# Autodesk Inventor assembly: Assembly2
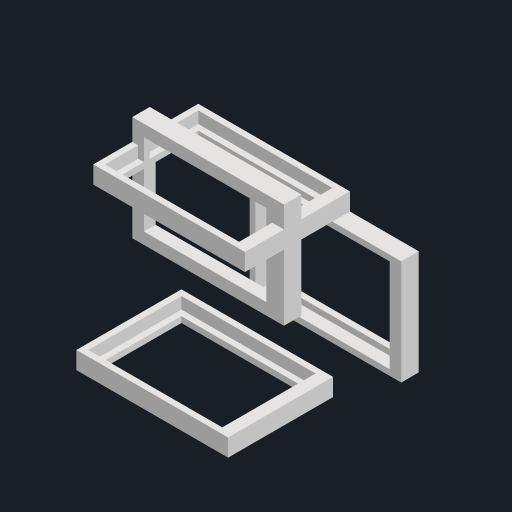
[picture p0: Inventor's stored thumbnail of the model, 512x512]
Saved by Autodesk Inventor 2024 (Build 280153000, 153)
## iProperties
Created: 2023-08-30
Part Number: Assembly2
Document SubType Name: Assembly
Designer: 91840
Author: 91840
## Documents named in this file (2)
- C:\Users\91840\Documents\Inventor\practice\project\DRAWINGS\Assembly2.iam
- C:\Users\91840\Documents\Inventor\practice\project\l.ipt
## Components (4 placed, 1 different names)
1. l:1 — Mate:1, Mate:2, Mate:3, Mate:4, Mate:5, Mate:6, Mate:10
2. l:2 — Mate:1, Mate:2, Mate:3, Mate:4
3. l:3 — Mate:5, Mate:6, Mate:7, Mate:8, Mate:9, Mate:10
4. l:4 — Mate:7, Mate:8, Mate:9
## Relationships (10: Mate 10)
- Mate:1: l:1 ↔ l:2
- Mate:2: l:1 ↔ l:2
- Mate:3: l:1 ↔ l:2
- Mate:4: l:1 ↔ l:2
- Mate:5: l:1 ↔ l:3
- Mate:6: l:1 ↔ l:3
- Mate:7: l:3 ↔ l:4
- Mate:8: l:3 ↔ l:4
- Mate:9: l:3 ↔ l:4
- Mate:10: l:1 ↔ l:3
